# Autodesk Inventor assembly: Assembly
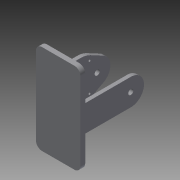
[picture p0: Inventor's stored thumbnail of the model, 180x180]
Saved by Autodesk Inventor 2015 (Build 190159000, 159)
## iProperties
Created: 2016-06-05
Part Number: Assembly
Document SubType Name: Assembly
Designer: EriveltonDell
Author: EriveltonDell
## Documents named in this file (4)
- C:\Users\EriveltonDell\Documents\Personal Projects\BB\Drawing\Assembly.iam
- C:\Users\EriveltonDell\Documents\Personal Projects\BB\Drawing\Base.ipt
- C:\Users\EriveltonDell\Documents\Personal Projects\BB\Drawing\Motor Support.ipt
- C:\Users\EriveltonDell\Documents\Personal Projects\BB\Drawing\Support.ipt
## Components (3 placed, 3 different names)
1. Base:1 — Flush:1, Mate:1, Mate:2, Mate:3, Mate:4, Flush:2
2. Motor Support:1 — Flush:1, Mate:1, Mate:2
3. Support:1 — Mate:3, Mate:4, Flush:2
## Relationships (6: Mate 4, Flush 2)
- Flush:1: Base:1 ↔ Motor Support:1
- Mate:1: Base:1 ↔ Motor Support:1
- Mate:2: Base:1 ↔ Motor Support:1
- Mate:3: Base:1 ↔ Support:1
- Mate:4: Base:1 ↔ Support:1
- Flush:2: Base:1 ↔ Support:1
